# Autodesk Inventor assembly: Сборка8
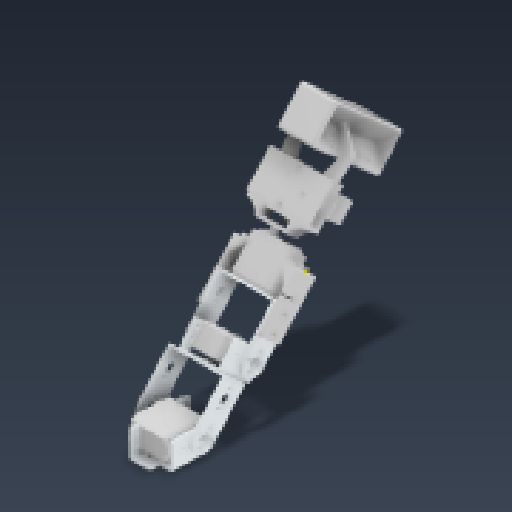
[picture p0: Inventor's stored thumbnail of the model, 512x512]
Saved by Autodesk Inventor 2025 (Build 290162000, 162)
## iProperties
Created: 2025-02-15
Part Number: Сборка8
Document SubType Name: Assembly
Designer: Phantom
Author: Phantom
## Documents named in this file (6)
- C:\Users\GameHD\Desktop\phantom 16950\Сборка8.iam
- C:\Users\GameHD\Desktop\phantom 16950\39593_txm-standard-scale pivot armwbearing.ipt
- C:\Users\GameHD\Desktop\phantom 16950\2000-0025-0002\2000-0025-0002_MIR4_MIR1_MIR.ipt
- C:\Users\GameHD\Desktop\phantom 16950\для захвата.ipt
- C:\Users\GameHD\Desktop\phantom 16950\39060_txm-standard servo bracket\39060_txm-standard servo bracket_MIR1.ipt
- C:\Users\GameHD\Desktop\phantom 16950\захват спереди.iam
## Components (10 placed, 5 different names)
1. 39593_txm-standard-scale pivot armwbearing:1 — Совмещение:1, Совмещение:2, Совмещение:3, Совмещение:4, Совмещение:6, Совмещение:8, Совмещение:17
2. 2000-0025-0002_MIR4_MIR1_MIR:1 — Совмещение:1, Совмещение:2, Совмещение:16, Совмещение:19
3. для захвата:1 — Совмещение:3, Совмещение:4, Совмещение:5
4. для захвата:2 — Совмещение:5, Совмещение:6
5. 39060_txm-standard servo bracket_MIR1:2 — Совмещение:8, Совмещение:9, Заподлицо:3, Совмещение:10, Совмещение:12, Заподлицо:5, Заподлицо:6, Совмещение:17
6. 2000-0025-0002_MIR4_MIR1_MIR:2 — Совмещение:9, Заподлицо:3, Совмещение:10
7. 39593_txm-standard-scale pivot armwbearing:2 — Совмещение:12, Заподлицо:5, Заподлицо:6, Совмещение:13, Совмещение:14, Совмещение:18
8. 39060_txm-standard servo bracket_MIR1:3 — Совмещение:13, Совмещение:14, Совмещение:15, Заподлицо:8, Совмещение:18
9. 2000-0025-0002_MIR4_MIR1_MIR:3 — Совмещение:15, Заподлицо:8
10. захват спереди:1 [sub-assembly] — Совмещение:16, Совмещение:19
## Relationships (22: Mate 18, Flush 4)
- Совмещение:1 [Mate]: 39593_txm-standard-scale pivot armwbearing:1 ↔ 2000-0025-0002_MIR4_MIR1_MIR:1
- Совмещение:2 [Mate]: 39593_txm-standard-scale pivot armwbearing:1 ↔ 2000-0025-0002_MIR4_MIR1_MIR:1
- Совмещение:3 [Mate]: 39593_txm-standard-scale pivot armwbearing:1 ↔ для захвата:1
- Совмещение:4 [Mate]: 39593_txm-standard-scale pivot armwbearing:1 ↔ для захвата:1
- Совмещение:5 [Mate]: для захвата:1 ↔ для захвата:2
- Совмещение:6 [Mate]: 39593_txm-standard-scale pivot armwbearing:1 ↔ для захвата:2
- Совмещение:8 [Mate]: 39593_txm-standard-scale pivot armwbearing:1 ↔ 39060_txm-standard servo bracket_MIR1:2
- Совмещение:9 [Mate]: 39060_txm-standard servo bracket_MIR1:2 ↔ 2000-0025-0002_MIR4_MIR1_MIR:2
- Заподлицо:3 [Flush] (1 mm): 39060_txm-standard servo bracket_MIR1:2 ↔ 2000-0025-0002_MIR4_MIR1_MIR:2
- Совмещение:10 [Mate]: 39060_txm-standard servo bracket_MIR1:2 ↔ 2000-0025-0002_MIR4_MIR1_MIR:2
- [Mate]: 39593_txm-standard-scale pivot armwbearing:2 ↔ 39060_txm-standard servo bracket_MIR1:3
- Совмещение:12 [Mate]: 39060_txm-standard servo bracket_MIR1:2 ↔ 39593_txm-standard-scale pivot armwbearing:2
- Заподлицо:5 [Flush] (14 mm): 39060_txm-standard servo bracket_MIR1:2 ↔ 39593_txm-standard-scale pivot armwbearing:2
- Заподлицо:6 [Flush] (-16 mm): 39060_txm-standard servo bracket_MIR1:2 ↔ 39593_txm-standard-scale pivot armwbearing:2
- Совмещение:13 [Mate]: 39593_txm-standard-scale pivot armwbearing:2 ↔ 39060_txm-standard servo bracket_MIR1:3
- Совмещение:14 [Mate] (-16 mm): 39593_txm-standard-scale pivot armwbearing:2 ↔ 39060_txm-standard servo bracket_MIR1:3
- Совмещение:15 [Mate]: 39060_txm-standard servo bracket_MIR1:3 ↔ 2000-0025-0002_MIR4_MIR1_MIR:3
- Заподлицо:8 [Flush] (3 mm): 39060_txm-standard servo bracket_MIR1:3 ↔ 2000-0025-0002_MIR4_MIR1_MIR:3
- Совмещение:16 [Mate]: 2000-0025-0002_MIR4_MIR1_MIR:1 ↔ захват спереди:1
- Совмещение:17 [Mate]: 39593_txm-standard-scale pivot armwbearing:1 ↔ 39060_txm-standard servo bracket_MIR1:2
- Совмещение:18 [Mate]: 39593_txm-standard-scale pivot armwbearing:2 ↔ 39060_txm-standard servo bracket_MIR1:3
- Совмещение:19 [Mate] (8 mm): 2000-0025-0002_MIR4_MIR1_MIR:1 ↔ захват спереди:1
## Named parameters: d19_d13 = 0 mm
